# Autodesk Inventor assembly: Assembly2
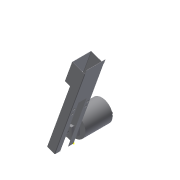
[picture p0: Inventor's stored thumbnail of the model, 180x180]
Saved by Autodesk Inventor 2019 (Build 230136000, 136)
## iProperties
Created: 2019-10-16
Part Number: Assembly2
Document SubType Name: Assembly
Designer: Admin
Author: Admin
## Documents named in this file (4)
- C:\Users\Admin\Documents\Assembly2.iam
- C:\Users\Admin\Documents\CAPPING SYSTEM DC MOTOR FIXING SYSTEM.ipt
- C:\Users\Admin\Documents\dc motor for capping system.ipt
- C:\Users\Admin\Documents\DC MOTOR NUT FOR CAPPING SYSTEM.ipt
## Components (4 placed, 3 different names)
1. CAPPING SYSTEM DC MOTOR FIXING SYSTEM:1 — Mate:1, Mate:2, Mate:4
2. dc motor for capping system:1 — Mate:1, Mate:2, Mate:3, Mate:5, Mate:6
3. DC MOTOR NUT FOR CAPPING SYSTEM:1 — Mate:5, Mate:6
4. DC MOTOR NUT FOR CAPPING SYSTEM:2 — Mate:3, Mate:4
## Relationships (6: Mate 6)
- Mate:1: CAPPING SYSTEM DC MOTOR FIXING SYSTEM:1 ↔ dc motor for capping system:1
- Mate:2 (10.16 mm): CAPPING SYSTEM DC MOTOR FIXING SYSTEM:1 ↔ dc motor for capping system:1
- Mate:3: dc motor for capping system:1 ↔ DC MOTOR NUT FOR CAPPING SYSTEM:2
- Mate:4: CAPPING SYSTEM DC MOTOR FIXING SYSTEM:1 ↔ DC MOTOR NUT FOR CAPPING SYSTEM:2
- Mate:5: dc motor for capping system:1 ↔ DC MOTOR NUT FOR CAPPING SYSTEM:1
- Mate:6: dc motor for capping system:1 ↔ DC MOTOR NUT FOR CAPPING SYSTEM:1
